# Autodesk Inventor assembly: Main
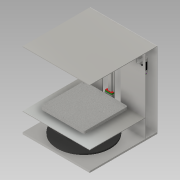
[picture p0: Inventor's stored thumbnail of the model, 180x180]
Saved by Autodesk Inventor 2016 (Build 200138000, 138)
## iProperties
Created: 2017-05-19
Part Number: Main
Document SubType Name: Assembly
Designer: 31745
Author: 31745
## Documents named in this file (11)
- H:\Projects\Printer #2\Printer2\IAM\Main.iam
- H:\Projects\Printer #2\Printer2\IPT\Machined Parts\Base Sheet.ipt
- H:\Projects\Printer #2\Printer2\IPT\Machined Parts\Print Bed.ipt
- H:\Projects\Printer #2\Printer2\IPT\Purchased Parts\M1173041- NEMA 17.ipt
- H:\Projects\Printer #2\Printer2\IPT\Purchased Parts\MGN Block.ipt
- H:\Projects\Printer #2\Printer2\IPT\Purchased Parts\MGN12.ipt
- H:\Projects\Printer #2\Printer2\IPT\Machined Parts\Interior Frame.ipt
- H:\Projects\Printer #2\Printer2\IPT\Machined Parts\Floor Sheet.ipt
- H:\Projects\Printer #2\Printer2\IPT\Machined Parts\Back Sheet.ipt
- H:\Projects\Printer #2\Printer2\IPT\Machined Parts\Ceiling.ipt
- H:\Projects\Printer #2\Printer2\IPT\Accessories\Spool Colorfabb.ipt
## Components (12 placed, 10 different names)
1. Base Sheet:1 — Flush:3, Mate:6, Flush:7, Flush:8, Flush:10, Mate:13, Flush:13, Flush:14, Mate:15
2. Print Bed:1 — Flush:4, Flush:5, Mate:4
3. MGN Block:1 — Mate:1, Mate:2, Flush:4
4. MGN12:1 — Mate:1, Mate:2, Flush:3, Flush:5, Mate:4, Mate:7, Mate:10
5. Interior Frame:1 — Mate:6, Flush:7, Mate:7, Mate:8, Flush:9, Mate:9, Mate:11, Mate:12, Flush:12
6. M1173041- NEMA 17:1 — Mate:8, Flush:8, Flush:9
7. Floor Sheet:1 — Mate:9, Flush:10, Mate:10, Mate:16
8. M1173041- NEMA 17:2 — Flush:11, Mate:11, Flush:12
9. M1173041- NEMA 17:3 — Flush:11, Mate:12
10. Back Sheet:1 — Mate:13, Flush:13, Flush:14, Flush:15, Flush:16, Mate:14
11. Ceiling:1 — Flush:15, Flush:16, Mate:14
12. Spool Colorfabb:1 — Mate:15, Mate:16
## Relationships (27: Mate 14, Flush 13)
- Mate:1: MGN Block:1 ↔ MGN12:1
- Mate:2: MGN Block:1 ↔ MGN12:1
- Flush:3 (121.0056 mm): Base Sheet:1 ↔ MGN12:1
- Flush:4 (2.54 mm): Print Bed:1 ↔ MGN Block:1
- Flush:5 (-76.5556 mm): Print Bed:1 ↔ MGN12:1
- Mate:4 (12.7 mm): Print Bed:1 ↔ MGN12:1
- Mate:6: Base Sheet:1 ↔ Interior Frame:1
- Flush:7: Base Sheet:1 ↔ Interior Frame:1
- Mate:7: MGN12:1 ↔ Interior Frame:1
- Mate:8: Interior Frame:1 ↔ M1173041- NEMA 17:1
- Flush:8: Base Sheet:1 ↔ M1173041- NEMA 17:1
- Flush:9: Interior Frame:1 ↔ M1173041- NEMA 17:1
- Mate:9: Interior Frame:1 ↔ Floor Sheet:1
- Flush:10: Base Sheet:1 ↔ Floor Sheet:1
- Mate:10: MGN12:1 ↔ Floor Sheet:1
- Flush:11: M1173041- NEMA 17:2 ↔ M1173041- NEMA 17:3
- Mate:11: Interior Frame:1 ↔ M1173041- NEMA 17:2
- Mate:12: Interior Frame:1 ↔ M1173041- NEMA 17:3
- Flush:12: Interior Frame:1 ↔ M1173041- NEMA 17:2
- Mate:13: Base Sheet:1 ↔ Back Sheet:1
- Flush:13: Base Sheet:1 ↔ Back Sheet:1
- Flush:14: Base Sheet:1 ↔ Back Sheet:1
- Flush:15: Back Sheet:1 ↔ Ceiling:1
- Flush:16: Back Sheet:1 ↔ Ceiling:1
- Mate:14: Back Sheet:1 ↔ Ceiling:1
- Mate:15 (6.35 mm): Base Sheet:1 ↔ Spool Colorfabb:1
- Mate:16 (6.35 mm): Floor Sheet:1 ↔ Spool Colorfabb:1
